# Autodesk Inventor assembly: FullLegAssembly
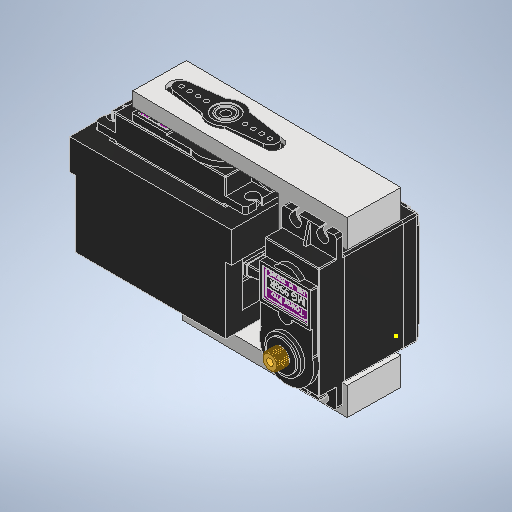
[picture p0: Inventor's stored thumbnail of the model, 512x512]
Saved by Autodesk Inventor 2025.1 (Build 291241020, 241B)
## iProperties
Created: 2024-09-10
Part Number: FullLegAssembly
Document SubType Name: Assembly
Designer: omiye
Author: omiye
## Documents named in this file (6)
- C:\Projects\Arduino\hexapod\legModels\FullLegAssembly.iam
- C:\Projects\Arduino\hexapod\legModels\MG996RServo.ipt
- C:\Projects\Arduino\hexapod\legModels\MG996RServoHolder.ipt
- C:\Projects\Arduino\hexapod\legModels\straightServoHorn.ipt
- C:\Users\omiye\Downloads\CHC M3 L18\CHC M3 L18.ipt
- C:\Projects\Arduino\hexapod\legModels\servoConnector.ipt
## Components (6 placed, 5 different names)
1. MG996RServo:1 — Mate:1, Mate:2, Mate:5, Mate:6, Mate:9, Mate:10, Mate:11, Mate:12
2. MG996RServoHolder:1 — Mate:1, Mate:2, Mate:7, Mate:8, Mate:9, Mate:10, Mate:11, Mate:12
3. straightServoHorn:1 — Mate:5, Mate:6, Mate:13, Mate:14, Mate:15
4. CHC M3 L18:1 — Mate:7, Mate:8
5. servoConnector:1 — Mate:13, Mate:14, Mate:15, Rigid:1, Mate:16
6. MG996RServo:2 — Rigid:1, Mate:16
## Relationships (15: Mate 14, WeldJoint 1)
- Mate:1: MG996RServo:1 ↔ MG996RServoHolder:1
- Mate:2: MG996RServo:1 ↔ MG996RServoHolder:1
- Mate:5: MG996RServo:1 ↔ straightServoHorn:1
- Mate:6: MG996RServo:1 ↔ straightServoHorn:1
- Mate:7: MG996RServoHolder:1 ↔ CHC M3 L18:1
- Mate:8: MG996RServoHolder:1 ↔ CHC M3 L18:1
- Mate:9: MG996RServo:1 ↔ MG996RServoHolder:1
- Mate:10: MG996RServo:1 ↔ MG996RServoHolder:1
- Mate:11: MG996RServo:1 ↔ MG996RServoHolder:1
- Mate:12: MG996RServo:1 ↔ MG996RServoHolder:1
- Mate:13: straightServoHorn:1 ↔ servoConnector:1
- Mate:14: straightServoHorn:1 ↔ servoConnector:1
- Mate:15: straightServoHorn:1 ↔ servoConnector:1
- Rigid:1 [WeldJoint]: servoConnector:1 ↔ MG996RServo:2
- Mate:16: servoConnector:1 ↔ MG996RServo:2
